# Autodesk Inventor assembly: motor_w_gear
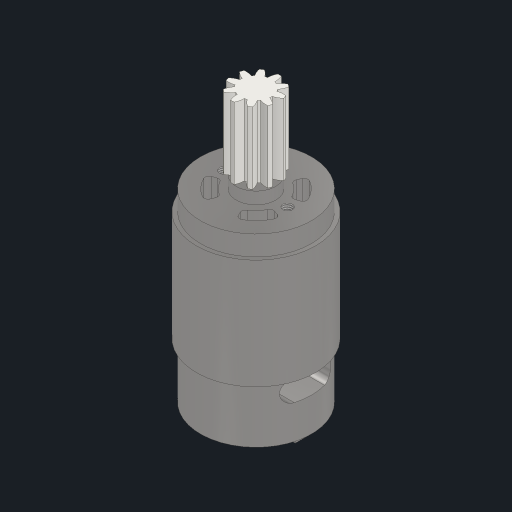
[picture p0: Inventor's stored thumbnail of the model, 512x512]
Saved by Autodesk Inventor 2023 (Build 270158000, 158)
## iProperties
Created: 2024-04-29
Part Number: motor_w_gear
Document SubType Name: Assembly
Designer: szymo
Mass: 122 g
Surface Area: 86.8548 cm^2
Volume: 30.5717 cm^3
Author: szymo
## Documents named in this file (3)
- D:\roboilo\robots\codename wafel - australia\3d_parts\rev4\motor_w_gear.iam
- D:\roboilo\robots\codename wafel - australia\3d_parts\rev4\rs390.ipt
- D:\roboilo\robots\codename wafel - australia\3d_parts\rev4\Design Accelerator\rs390_gear.iam
## Components (2 placed, 2 different names)
1. rs390_gear:1 [sub-assembly] — Mate:1, Mate:2
2. rs390:1 — Mate:1, Mate:2
## Relationships (2: Mate 2)
- Mate:1: rs390_gear:1 ↔ rs390:1
- Mate:2 (1 mm): rs390_gear:1 ↔ rs390:1
